# Autodesk Inventor assembly: Case and Top Assembly
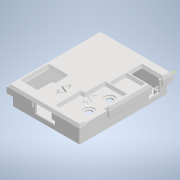
[picture p0: Inventor's stored thumbnail of the model, 180x180]
Saved by Autodesk Inventor 2020 (Build 240168000, 168)
## iProperties
Created: 2020-05-28
Part Number: Case and Top Assembly
Document SubType Name: Assembly
Designer: maple
Author: maple
## Documents named in this file (3)
- C:\Nitro\Github\Air-Conditioner\Air_Conditioner\SubParts\3D\Case and Top Assembly.iam
- C:\Nitro\Github\Air-Conditioner\Air_Conditioner\SubParts\3D\Mainboard_Case_LOGO.ipt
- C:\Nitro\Github\Air-Conditioner\Air_Conditioner\SubParts\3D\Mainboard_Case_Top.ipt
## Components (2 placed, 2 different names)
1. Mainboard_Case_LOGO:1 — Mate:1, Mate:2
2. Mainboard_Case_Top:1 — Mate:1, Mate:2
## Relationships (2: Mate 2)
- Mate:1 (1 mm): Mainboard_Case_LOGO:1 ↔ Mainboard_Case_Top:1
- Mate:2 (1 mm): Mainboard_Case_LOGO:1 ↔ Mainboard_Case_Top:1
